# Autodesk Inventor assembly: gyroPhone01
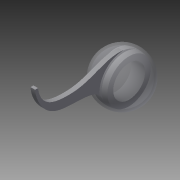
[picture p0: Inventor's stored thumbnail of the model, 180x180]
Saved by Autodesk Inventor 2013 (Build 170138000, 138)
## iProperties
Created: 2013-01-08
Part Number: gyroPhone01
Document SubType Name: Assembly
Designer: Nano
Author: Nano
## Documents named in this file (4)
- C:\Users\Nano\Documents\InventorByron\InventorMasterProject\gyroPhone01\gyroPhone01.iam
- C:\Users\Nano\Documents\InventorByron\InventorMasterProject\gyroPhone01\bodySphere.ipt
- C:\Users\Nano\Documents\InventorByron\InventorMasterProject\gyroPhone01\bigWheel.ipt
- C:\Users\Nano\Documents\InventorByron\InventorMasterProject\gyroPhone01\bodyMainAirPipe.ipt
## Components (3 placed, 3 different names)
1. bodySphere:1
2. bigWheel:1
3. bodyMainAirPipe:1 — Flush:1
## Relationships (1: Flush 1)
- Flush:1: bodyMainAirPipe:1
